# Autodesk Inventor assembly: M178-PHTM-3000-05
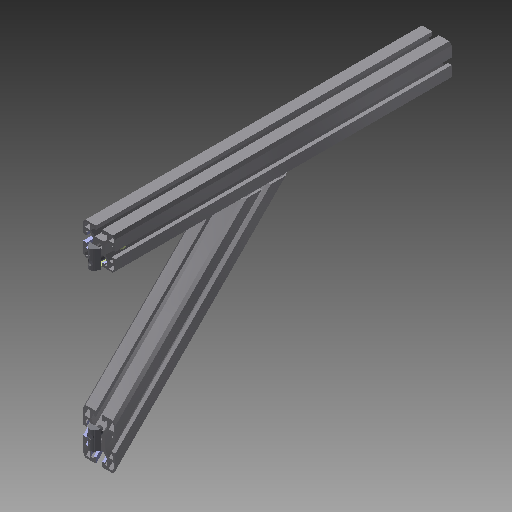
[picture p0: Inventor's stored thumbnail of the model, 512x512]
Saved by Autodesk Inventor 2018 (Build 220105000, 105)
## iProperties
Created: 2004-11-24
Part Number: M178-PHTM-3000-05
Document SubType Name: Assembly
Designer: Autodesk, Inc.
Manufacturer: Standard
Standards Organization: Custom
Description: PHANTOM, HUTCH OVERHANG
Mass: 1298.12 g
Surface Area: 3322.23 cm^2
Volume: 458.284 cm^3
Density: 2.83257 g/cm^3
CAGE: 1LJX3
Dept. ID: Product Design
Description #2: ---
Finish #1: ---
Finish #2: ---
Material ID: ---
Project Number: ---
Author: Autodesk, Inc.
## Documents named in this file (9)
- C:\Autodesk\autodesk_inventor_2017_samples\Models\Assemblies\Test Station\Components\M178-3000 Overhange Phantom.iam
- C:\Autodesk\autodesk_inventor_2017_samples\Models\Assemblies\Test Station\Components\M178-3003.ipt
- C:\Autodesk\autodesk_inventor_2017_samples\Models\Assemblies\Test Station\Components\M178-3004.ipt
- C:\Autodesk\autodesk_inventor_2017_samples\Models\Assemblies\Test Station\Components\20-004.iam
- C:\Autodesk\autodesk_inventor_2017_samples\Models\Assemblies\Test Station\Components\20-058.ipt
- C:\Autodesk\autodesk_inventor_2017_samples\Models\Assemblies\Test Station\Components\24-120-8.ipt
- C:\Users\kelleyb.ADS\Desktop\Samples MIGRATED 2009 224 RTM_1\Standard Parts\Test Station Content\Extrusions\40 Series Profiles.ipt
- C:\Users\kelleyb.ADS\Desktop\Samples MIGRATED 2009 224 RTM_1\Standard Parts\Test Station Content\Fastners\2X-YYY-ZZ IPS Screws.ipt
- C:\Users\kelleyb.ADS\Desktop\Samples MIGRATED 2009 224 RTM_1\Standard Parts\Test Station Content\Fastners\20-XXX TSlot Nuts.ipt
## Components (7 placed, 5 different names)
1. M178-3003:1 — Insert:1, Angle:1, Mate:1, Flush:1, Flush:2
2. M178-3004:2 — Mate:1, Flush:1, Flush:2, Insert:2, Insert:3, Mate:3, Mate:4, Angle:2, Angle:3
3. 20-004:1 [sub-assembly] — Insert:1, Angle:1
4. 24-120-8:1 — Insert:2, Mate:2
5. 24-120-8:2 — Insert:3, Mate:5
6. 20-058:1 — Mate:2, Mate:3, Angle:3
7. 20-058:2 — Mate:4, Mate:5, Angle:2
## Relationships (13: Mate 5, Insert 3, Angle 3, Flush 2)
- Insert:1: M178-3003:1 ↔ 20-004:1
- Angle:1 (0 deg): M178-3003:1 ↔ 20-004:1
- Mate:1: M178-3003:1 ↔ M178-3004:2
- Flush:1: M178-3003:1 ↔ M178-3004:2
- Flush:2: M178-3003:1 ↔ M178-3004:2
- Insert:2: M178-3004:2 ↔ 24-120-8:1
- Insert:3: M178-3004:2 ↔ 24-120-8:2
- Mate:2: 24-120-8:1 ↔ 20-058:1
- Mate:3 (4.5 mm): M178-3004:2 ↔ 20-058:1
- Mate:4 (4.5 mm): M178-3004:2 ↔ 20-058:2
- Mate:5: 24-120-8:2 ↔ 20-058:2
- Angle:2 (0 deg): M178-3004:2 ↔ 20-058:2
- Angle:3 (0 deg): M178-3004:2 ↔ 20-058:1
